# Autodesk Inventor assembly: hipjoint
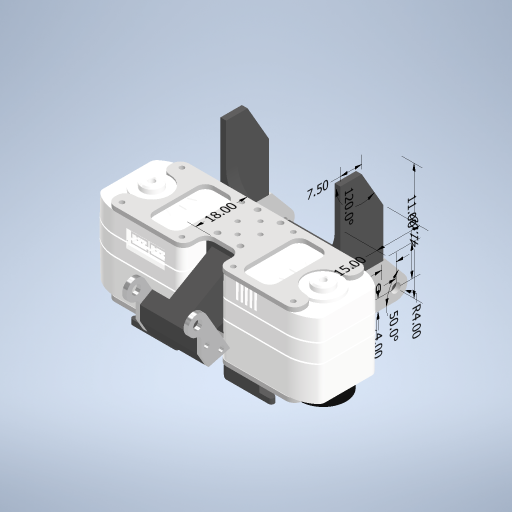
[picture p0: Inventor's stored thumbnail of the model, 512x512]
Saved by Autodesk Inventor 2024.1 (Build 281209000, 209)
## iProperties
Created: 2024-10-09
Part Number: hipjoint
Document SubType Name: Assembly
Designer: hibik
Author: hibik
## Documents named in this file (8)
- C:\Users\hibik\Documents\Robomech\HR\Eglantyne\hard\under_body\hipjoint.iam
- C:\Users\hibik\Documents\Robomech\HR\Eglantyne\hard\under_body\hipjoint_upper.ipt
- C:\Users\hibik\Documents\Robomech\HR\Eglantyne\hard\needed_model\KRS3300モータ.ipt
- C:\Users\hibik\Documents\Robomech\HR\Eglantyne\hard\needed_model\KRS3300サーボホーン.ipt
- C:\Users\hibik\Documents\Robomech\HR\Eglantyne\hard\under_body\hipjoint_middle.ipt
- C:\Users\hibik\Documents\Robomech\HR\Eglantyne\hard\under_body\board_setter_joint.ipt
- C:\Users\hibik\Documents\Robomech\HR\Eglantyne\hard\under_body\joit_cover_hip.ipt
- C:\Users\hibik\Documents\Robomech\HR\Eglantyne\hard\under_body\battery_cover_setter_joint.ipt
## Components (13 placed, 7 different names)
1. hipjoint_upper:1 — 挿入:1, 挿入:2, 角度:2, メイト:1, フラッシュ:1, メイト:2
2. KRS3300モータ:1 — 挿入:1, 角度:1, 挿入:3, 挿入:5, 挿入:6
3. KRS3300モータ:2 — 挿入:2, 角度:1, 角度:2, 挿入:4, メイト:5
4. KRS3300サーボホーン:1 — 挿入:4
5. KRS3300サーボホーン:2 — 挿入:3
6. hipjoint_middle:1 — メイト:1, フラッシュ:1, メイト:2, メイト:3, フラッシュ:2, フラッシュ:3, メイト:4, フラッシュ:4, フラッシュ:5, フラッシュ:6, フラッシュ:7, メイト:6, メイト:7, フラッシュ:8, フラッシュ:9
7. board_setter_joint:1 — メイト:3, フラッシュ:2, フラッシュ:3
8. board_setter_joint:2 — メイト:4, フラッシュ:4, フラッシュ:5
9. hipjoint_upper:2 — メイト:5, 挿入:5, 挿入:6, 挿入:7, 挿入:8, 挿入:9, 挿入:10
10. joit_cover_hip:1 — 挿入:7, 挿入:8
11. joit_cover_hip:2 — 挿入:9, 挿入:10
12. battery_cover_setter_joint:1 — フラッシュ:6, フラッシュ:7, メイト:6
13. battery_cover_setter_joint:2 — メイト:7, フラッシュ:8, フラッシュ:9
## Relationships (28: Insert 10, Flush 9, Mate 7, Angle 2)
- 挿入:1 [Insert]: hipjoint_upper:1 ↔ KRS3300モータ:1
- 挿入:2 [Insert]: hipjoint_upper:1 ↔ KRS3300モータ:2
- 角度:1 [Angle] (180 deg): KRS3300モータ:1 ↔ KRS3300モータ:2
- 角度:2 [Angle] (0 deg): hipjoint_upper:1 ↔ KRS3300モータ:2
- 挿入:3 [Insert]: KRS3300モータ:1 ↔ KRS3300サーボホーン:2
- 挿入:4 [Insert]: KRS3300モータ:2 ↔ KRS3300サーボホーン:1
- メイト:1 [Mate]: hipjoint_upper:1 ↔ hipjoint_middle:1
- フラッシュ:1 [Flush]: hipjoint_upper:1 ↔ hipjoint_middle:1
- メイト:2 [Mate]: hipjoint_upper:1 ↔ hipjoint_middle:1
- メイト:3 [Mate]: hipjoint_middle:1 ↔ board_setter_joint:1
- フラッシュ:2 [Flush]: hipjoint_middle:1 ↔ board_setter_joint:1
- フラッシュ:3 [Flush]: hipjoint_middle:1 ↔ board_setter_joint:1
- メイト:4 [Mate]: hipjoint_middle:1 ↔ board_setter_joint:2
- フラッシュ:4 [Flush]: hipjoint_middle:1 ↔ board_setter_joint:2
- フラッシュ:5 [Flush]: hipjoint_middle:1 ↔ board_setter_joint:2
- メイト:5 [Mate]: KRS3300モータ:2 ↔ hipjoint_upper:2
- 挿入:5 [Insert]: KRS3300モータ:1 ↔ hipjoint_upper:2
- 挿入:6 [Insert]: KRS3300モータ:1 ↔ hipjoint_upper:2
- 挿入:7 [Insert]: hipjoint_upper:2 ↔ joit_cover_hip:1
- 挿入:8 [Insert]: hipjoint_upper:2 ↔ joit_cover_hip:1
- 挿入:9 [Insert]: hipjoint_upper:2 ↔ joit_cover_hip:2
- 挿入:10 [Insert]: hipjoint_upper:2 ↔ joit_cover_hip:2
- フラッシュ:6 [Flush]: hipjoint_middle:1 ↔ battery_cover_setter_joint:1
- フラッシュ:7 [Flush]: hipjoint_middle:1 ↔ battery_cover_setter_joint:1
- メイト:6 [Mate]: hipjoint_middle:1 ↔ battery_cover_setter_joint:1
- メイト:7 [Mate]: hipjoint_middle:1 ↔ battery_cover_setter_joint:2
- フラッシュ:8 [Flush]: hipjoint_middle:1 ↔ battery_cover_setter_joint:2
- フラッシュ:9 [Flush]: hipjoint_middle:1 ↔ battery_cover_setter_joint:2
